# Autodesk Inventor assembly: FocuserAssembly
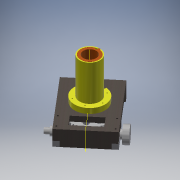
[picture p0: Inventor's stored thumbnail of the model, 180x180]
Saved by Autodesk Inventor 2019.3 (Build 233278000, 278)
## iProperties
Created: 2019-01-19
Part Number: FocuserAssembly
Document SubType Name: Assembly
Designer: steele
Author: steele
## Documents named in this file (7)
- C:\git\CAD-Development\robSteele\ShapeWays\TelescopeProjects\Focuser\FocuserAssembly.iam
- C:\git\CAD-Development\robSteele\ShapeWays\TelescopeProjects\Focuser\ExternalStationaryOuterRing.ipt
- C:\git\CAD-Development\robSteele\ShapeWays\TelescopeProjects\Focuser\InnerThreadedFocusTube.ipt
- C:\git\CAD-Development\robSteele\ShapeWays\TelescopeProjects\Focuser\WormDrive02.iam
- C:\git\CAD-Development\robSteele\ShapeWays\TelescopeProjects\Focuser\SupportForAxel.ipt
- C:\git\CAD-Development\robSteele\ShapeWays\TelescopeProjects\Focuser\HoldWormDrive.ipt
- C:\git\CAD-Development\robSteele\ShapeWays\TelescopeProjects\Focuser\HoldWormDrive_MIR.ipt
## Components (6 placed, 6 different names)
1. ExternalStationaryOuterRing:1 — Insert:1, Mate:1, Insert:2
2. InnerThreadedFocusTube:1 — Insert:1, Mate:1
3. WormDrive02:1 [sub-assembly] — Mate:2
4. SupportForAxel:1 — Insert:2, Mate:2, Mate:4, Flush:3, Flush:4
5. HoldWormDrive:2 — Mate:4, Flush:3, Flush:4
6. HoldWormDrive_MIR:1
## Relationships (7: Mate 3, Insert 2, Flush 2)
- Insert:1: ExternalStationaryOuterRing:1 ↔ InnerThreadedFocusTube:1
- Mate:1: ExternalStationaryOuterRing:1 ↔ InnerThreadedFocusTube:1
- Insert:2: ExternalStationaryOuterRing:1 ↔ SupportForAxel:1
- Mate:2: WormDrive02:1 ↔ SupportForAxel:1
- Mate:4: SupportForAxel:1 ↔ HoldWormDrive:2
- Flush:3: SupportForAxel:1 ↔ HoldWormDrive:2
- Flush:4: SupportForAxel:1 ↔ HoldWormDrive:2
## Named parameters: mateToStationaryTube = 0 mm
